# Autodesk Inventor assembly: montagem
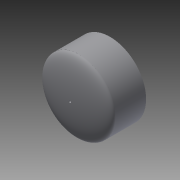
[picture p0: Inventor's stored thumbnail of the model, 180x180]
Saved by Autodesk Inventor 2015 (Build 190159000, 159)
## iProperties
Created: 2019-09-28
Part Number: montagem
Document SubType Name: Assembly
Designer: gabri
Author: gabri
## Documents named in this file (3)
- C:\Users\gabri\Documents\Inventor\cansat-3d\montagem.iam
- C:\Users\gabri\Documents\Inventor\cansat-3d\data_logger.ipt
- C:\Users\gabri\Documents\Inventor\cansat-3d\cup.ipt
## Components (2 placed, 2 different names)
1. data_logger:1 — Insert:1
2. cup:1 — Insert:1
## Relationships (1: Insert 1)
- Insert:1: data_logger:1 ↔ cup:1
